# Autodesk Inventor assembly: ASY дренаж угольные
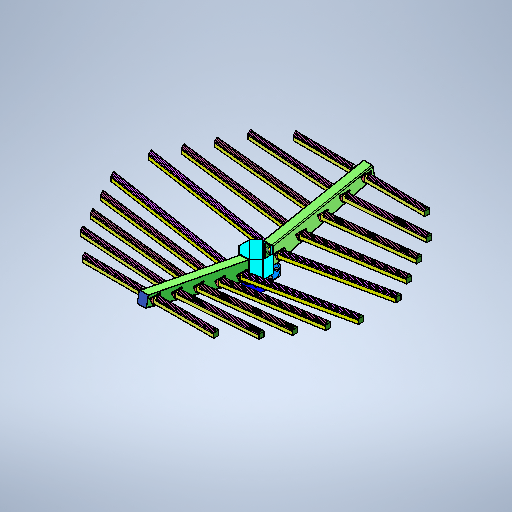
[picture p0: Inventor's stored thumbnail of the model, 512x512]
Saved by Autodesk Inventor 2025.1 (Build 291241020, 241B)
## iProperties
Created: 2024-12-09
Part Number: ASY дренаж угольные
Document SubType Name: Assembly
Designer: user
Author: user
## Documents named in this file (20)
- C:\Users\user\YandexDisk-badmisterfox\home pc\Inventor\Manturovo\Manturovo_Se-clar\Дренаж на угольные\2200\ASY BOTTOM filter distribution system.iam
- C:\Users\user\YandexDisk-badmisterfox\home pc\Inventor\Manturovo\Manturovo_Se-clar\Дренаж на угольные\2200\drain flange.ipt
- C:\Users\user\YandexDisk-badmisterfox\home pc\Inventor\Manturovo\Manturovo_Se-clar\Дренаж на угольные\2200\dished head.ipt
- C:\Users\user\YandexDisk-badmisterfox\home pc\Inventor\Manturovo\Manturovo_Se-clar\Дренаж на угольные\2200\DSB-102 ridge bottom.ipt
- C:\Users\user\YandexDisk-badmisterfox\home pc\Inventor\Manturovo\Manturovo_Se-clar\Дренаж на угольные\2200\DSB-101 Axis.ipt
- C:\Users\user\YandexDisk-badmisterfox\home pc\Inventor\Manturovo\Manturovo_Se-clar\Дренаж на угольные\2200\DSB-104 ridge end cap.ipt
- C:\Users\user\YandexDisk-badmisterfox\home pc\Inventor\Manturovo\Manturovo_Se-clar\Дренаж на угольные\2200\DSB-103 Ridge top.ipt
- C:\Users\user\YandexDisk-badmisterfox\home pc\Inventor\Manturovo\Manturovo_Se-clar\Дренаж на угольные\2200\ASY DSB beam 1.iam
- C:\Users\user\YandexDisk-badmisterfox\home pc\Inventor\Manturovo\Manturovo_Se-clar\Дренаж на угольные\2200\000 DSB dimentions.ipt
- C:\Users\user\YandexDisk-badmisterfox\home pc\Inventor\Manturovo\Manturovo_Se-clar\Дренаж на угольные\2200\DSB 111 outer tube.ipt
- C:\Users\user\YandexDisk-badmisterfox\home pc\Inventor\Manturovo\Manturovo_Se-clar\Дренаж на угольные\2200\DSB 110 drain sustem flange.ipt
- C:\Users\user\YandexDisk-badmisterfox\home pc\Inventor\Manturovo\Manturovo_Se-clar\Дренаж на угольные\2200\ASY DS-B beam 2.iam
- C:\Users\user\YandexDisk-badmisterfox\home pc\Inventor\Manturovo\Manturovo_Se-clar\Дренаж на угольные\2200\ASY DS-B beam 3.iam
- C:\Users\user\YandexDisk-badmisterfox\home pc\Inventor\Manturovo\Manturovo_Se-clar\Дренаж на угольные\2200\ASY DS-B beam 4.iam
- C:\Users\user\YandexDisk-badmisterfox\home pc\Inventor\Manturovo\Manturovo_Se-clar\Дренаж на угольные\2200\DSB 210 Axis cap.ipt
- C:\Users\user\YandexDisk-badmisterfox\home pc\Inventor\Manturovo\Content Center Files\en-US\SS-ISO 4017\ISO 4017 - M10 x 100SS-ISO.ipt
- C:\Users\user\YandexDisk-badmisterfox\home pc\Inventor\Manturovo\Content Center Files\en-US\SS-ISO 4032\ISO 4032 - M10SS-ISO.ipt
- C:\Users\user\YandexDisk-badmisterfox\home pc\Inventor\Manturovo\Manturovo_Se-clar\Дренаж на угольные\2200\ASY DS-B beam 45.iam
- C:\Users\user\YandexDisk-badmisterfox\home pc\Inventor\Manturovo\Content Center Files\en-US\ISO 7005-1 01 - PN 10\ISO 7005-1 Plate Flange for Welding Type 01 Flat Face - ISO PN 10 DN150.ipt
- C:\Users\user\YandexDisk-badmisterfox\home pc\Inventor\Manturovo\Content Center Files\en-US\ISO 8676(2)\ISO 8676 - M16 x 1.5 x 35 - ISO.ipt
## Components (47 placed, 19 different names)
1. 000 DSB dimentions:1
2. dished head:1 — Mate:4, Flush:3, Flush:4, Rigid:36
3. DSB-102 ridge bottom:1 — Mate:10, Mate:11, Flush:5, Rigid:63, Rigid:66, Rigid:68, Rigid:70, Rigid:72
4. drain flange:1 — Rigid:37, Rigid:73
5. DSB-101 Axis:1 — Mate:16, Mate:19, Mate:22, Flush:7, Flush:9, Mate:27
6. DSB-101 Axis:2 — Mate:11, Mate:21, Mate:23, Mate:24, Mate:25, Flush:8, Mate:26
7. DSB-102 ridge bottom:2 — Mate:15, Mate:16, Flush:6, Rigid:53, Rigid:54, Rigid:55, Rigid:56, Rigid:61, Mate:27
8. DSB-104 ridge end cap:1 — Rigid:51
9. DSB-104 ridge end cap:2 — Rigid:52
10. DSB-103 Ridge top:1 — Mate:20, Mate:21, Flush:5, Rigid:51, Rigid:62, Rigid:64, Rigid:65, Rigid:67, Rigid:69, Mate:26
11. ASY DSB beam 1:1 [sub-assembly] — Rigid:72
12. DSB 111 outer tube:1 — Rigid:36, Rigid:37
13. DSB 110 drain sustem flange:1 — Mate:10, Mate:15, Mate:18, Mate:20, Mate:22, Mate:23, Insert:1, Insert:2, Insert:3, Insert:4, Insert:5, Insert:6, Flush:8, Flush:9
14. ASY DS-B beam 2:1 [sub-assembly] — Rigid:70
15. ASY DS-B beam 3:1 [sub-assembly] — Rigid:68
16. ASY DS-B beam 4:1 [sub-assembly] — Rigid:66
17. DSB-103 Ridge top:2 — Mate:18, Mate:19, Flush:6, Rigid:52, Rigid:57, Rigid:58, Rigid:59, Rigid:60, Rigid:71
18. DSB 210 Axis cap:1 — Mate:25
19. ASY DSB beam 1:2 [sub-assembly] — Rigid:62
20. ASY DSB beam 1:3 [sub-assembly] — Rigid:53, Rotational:4, Rotational:5, Rotational:6
21. ASY DSB beam 1:4 [sub-assembly] — Rigid:57, Rotational:1, Rotational:2, Rotational:3
22. ASY DS-B beam 2:2 [sub-assembly] — Rigid:69
23. ASY DS-B beam 3:2 [sub-assembly] — Rigid:67
24. ASY DS-B beam 4:2 [sub-assembly] — Rigid:65
25. ASY DS-B beam 2:3 [sub-assembly] — Rigid:54
26. ASY DS-B beam 3:3 [sub-assembly] — Rigid:55
27. ASY DS-B beam 4:3 [sub-assembly] — Rigid:56
28. ASY DS-B beam 2:4 [sub-assembly] — Rigid:58
29. ASY DS-B beam 3:4 [sub-assembly] — Rigid:59
30. ASY DS-B beam 4:4 [sub-assembly] — Rigid:60
31. ISO 4017 - M10 x 100:1 — Rotational:1
32. ISO 4017 - M10 x 100:2 — Rotational:3
33. ISO 4017 - M10 x 100:3 — Rotational:2
34. ISO 4032 - M10:1 — Rotational:4
35. ISO 4032 - M10:2 — Rotational:5
36. ISO 4032 - M10:3 — Rotational:6
37. ASY DS-B beam 45:1 [sub-assembly] — Rigid:61
38. ASY DS-B beam 45:2 [sub-assembly] — Rigid:71
39. ASY DS-B beam 45:3 [sub-assembly] — Rigid:64
40. ASY DS-B beam 45:4 [sub-assembly] — Rigid:63
41. ISO 7005-1 Plate Flange for Welding Type 01 Flat Face - ISO PN 10 DN150:1 — Rigid:73
42. ISO 8676 M16 x 1.5 x 35:1 — Insert:1
43. ISO 8676 M16 x 1.5 x 35:2 — Insert:2
44. ISO 8676 M16 x 1.5 x 35:3 — Insert:3
45. ISO 8676 M16 x 1.5 x 35:4 — Insert:4
46. ISO 8676 M16 x 1.5 x 35:5 — Insert:5
47. ISO 8676 M16 x 1.5 x 35:6 — Insert:6
## Relationships (59: WeldJoint 25, Mate 15, Flush 7, RevoluteJoint 6, Insert 6)
- Mate:4: dished head:1
- Flush:3: dished head:1
- Flush:4: dished head:1
- Rigid:36 [WeldJoint]: dished head:1 ↔ DSB 111 outer tube:1
- Rigid:37 [WeldJoint]: drain flange:1 ↔ DSB 111 outer tube:1
- Mate:10: DSB-102 ridge bottom:1 ↔ DSB 110 drain sustem flange:1
- Mate:11: DSB-102 ridge bottom:1 ↔ DSB-101 Axis:2
- Mate:15: DSB-102 ridge bottom:2 ↔ DSB 110 drain sustem flange:1
- Mate:16: DSB-101 Axis:1 ↔ DSB-102 ridge bottom:2
- Mate:18: DSB 110 drain sustem flange:1 ↔ DSB-103 Ridge top:2
- Mate:19: DSB-101 Axis:1 ↔ DSB-103 Ridge top:2
- Mate:20: DSB-103 Ridge top:1 ↔ DSB 110 drain sustem flange:1
- Mate:21: DSB-101 Axis:2 ↔ DSB-103 Ridge top:1
- Flush:5: DSB-102 ridge bottom:1 ↔ DSB-103 Ridge top:1
- Flush:6: DSB-102 ridge bottom:2 ↔ DSB-103 Ridge top:2
- Rigid:51 [WeldJoint]: DSB-104 ridge end cap:1 ↔ DSB-103 Ridge top:1
- Rigid:52 [WeldJoint]: DSB-104 ridge end cap:2 ↔ DSB-103 Ridge top:2
- Rigid:53 [WeldJoint]: DSB-102 ridge bottom:2 ↔ ASY DSB beam 1:3
- Rigid:54 [WeldJoint]: DSB-102 ridge bottom:2 ↔ ASY DS-B beam 2:3
- Rigid:55 [WeldJoint]: DSB-102 ridge bottom:2 ↔ ASY DS-B beam 3:3
- Rigid:56 [WeldJoint]: DSB-102 ridge bottom:2 ↔ ASY DS-B beam 4:3
- Rigid:57 [WeldJoint]: DSB-103 Ridge top:2 ↔ ASY DSB beam 1:4
- Rigid:58 [WeldJoint]: DSB-103 Ridge top:2 ↔ ASY DS-B beam 2:4
- Rigid:59 [WeldJoint]: DSB-103 Ridge top:2 ↔ ASY DS-B beam 3:4
- Rigid:60 [WeldJoint]: DSB-103 Ridge top:2 ↔ ASY DS-B beam 4:4
- Rotational:1 [RevoluteJoint]: ASY DSB beam 1:4 ↔ ISO 4017 - M10 x 100:1
- Rotational:2 [RevoluteJoint]: ASY DSB beam 1:4 ↔ ISO 4017 - M10 x 100:3
- Rotational:3 [RevoluteJoint]: ASY DSB beam 1:4 ↔ ISO 4017 - M10 x 100:2
- Rotational:4 [RevoluteJoint]: ASY DSB beam 1:3 ↔ ISO 4032 - M10:1
- Rotational:5 [RevoluteJoint]: ASY DSB beam 1:3 ↔ ISO 4032 - M10:2
- Rotational:6 [RevoluteJoint]: ASY DSB beam 1:3 ↔ ISO 4032 - M10:3
- Rigid:61 [WeldJoint]: DSB-102 ridge bottom:2 ↔ ASY DS-B beam 45:1
- Rigid:62 [WeldJoint]: DSB-103 Ridge top:1 ↔ ASY DSB beam 1:2
- Rigid:63 [WeldJoint]: DSB-102 ridge bottom:1 ↔ ASY DS-B beam 45:4
- Rigid:64 [WeldJoint]: DSB-103 Ridge top:1 ↔ ASY DS-B beam 45:3
- Rigid:65 [WeldJoint]: DSB-103 Ridge top:1 ↔ ASY DS-B beam 4:2
- Rigid:66 [WeldJoint]: DSB-102 ridge bottom:1 ↔ ASY DS-B beam 4:1
- Rigid:67 [WeldJoint]: DSB-103 Ridge top:1 ↔ ASY DS-B beam 3:2
- Rigid:68 [WeldJoint]: DSB-102 ridge bottom:1 ↔ ASY DS-B beam 3:1
- Rigid:69 [WeldJoint]: DSB-103 Ridge top:1 ↔ ASY DS-B beam 2:2
- Rigid:70 [WeldJoint]: DSB-102 ridge bottom:1 ↔ ASY DS-B beam 2:1
- Rigid:71 [WeldJoint]: DSB-103 Ridge top:2 ↔ ASY DS-B beam 45:2
- Rigid:72 [WeldJoint]: DSB-102 ridge bottom:1 ↔ ASY DSB beam 1:1
- Rigid:73 [WeldJoint]: drain flange:1 ↔ ISO 7005-1 Plate Flange for Welding Type 01 Flat Face - ISO PN 10 DN150:1
- Mate:22: DSB-101 Axis:1 ↔ DSB 110 drain sustem flange:1
- Mate:23: DSB-101 Axis:2 ↔ DSB 110 drain sustem flange:1
- Flush:7: DSB-101 Axis:1
- Mate:24: DSB-101 Axis:2
- Insert:1: DSB 110 drain sustem flange:1 ↔ ISO 8676 M16 x 1.5 x 35:1
- Insert:2: DSB 110 drain sustem flange:1 ↔ ISO 8676 M16 x 1.5 x 35:2
- Insert:3: DSB 110 drain sustem flange:1 ↔ ISO 8676 M16 x 1.5 x 35:3
- Insert:4: DSB 110 drain sustem flange:1 ↔ ISO 8676 M16 x 1.5 x 35:4
- Insert:5: DSB 110 drain sustem flange:1 ↔ ISO 8676 M16 x 1.5 x 35:5
- Insert:6: DSB 110 drain sustem flange:1 ↔ ISO 8676 M16 x 1.5 x 35:6
- Mate:25: DSB-101 Axis:2 ↔ DSB 210 Axis cap:1
- Flush:8: DSB-101 Axis:2 ↔ DSB 110 drain sustem flange:1
- Flush:9: DSB-101 Axis:1 ↔ DSB 110 drain sustem flange:1
- Mate:26: DSB-101 Axis:2 ↔ DSB-103 Ridge top:1
- Mate:27: DSB-101 Axis:1 ↔ DSB-102 ridge bottom:2
